# Autodesk Inventor assembly: 조립
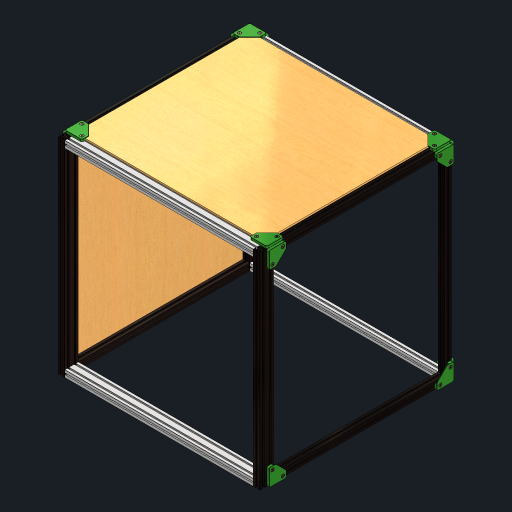
[picture p0: Inventor's stored thumbnail of the model, 512x512]
Saved by Autodesk Inventor 2024.1 (Build 281209000, 209)
## iProperties
Created: 2024-01-11
Part Number: 조립
Document SubType Name: Assembly
Designer: KBU
Author: KBU
## Documents named in this file (9)
- C:\Users\likek\Videos\Modeling\챔버\조립.iam
- C:\Users\likek\Videos\Modeling\챔버\600mm 20x20 Profile.ipt
- C:\Users\likek\Videos\Modeling\챔버\600mm 20x40 profile.ipt
- C:\Users\likek\Videos\Modeling\챔버\500mm 20x20 Profile.ipt
- C:\Users\likek\Videos\Modeling\챔버\모서리 결합 조립.iam
- C:\Users\likek\Videos\Modeling\챔버\510x570 패널.ipt
- C:\Users\likek\Videos\Modeling\챔버\550mm 20x40 profile.ipt
- C:\Users\likek\Videos\Modeling\챔버\550mm 20x20 Profile.ipt
- C:\Users\likek\Videos\Modeling\챔버\550x510 패널.ipt
## Components (31 placed, 8 different names)
1. 600mm 20x40 profile:1 — 플러쉬:12, 메이트:8, 플러쉬:13, 메이트:13, 플러쉬:23, 플러쉬:24, 메이트:46, 플러쉬:58, 플러쉬:59, 플러쉬:62, 플러쉬:63
2. 600mm 20x40 profile:2 — 플러쉬:6, 메이트:5, 플러쉬:7, 메이트:14, 메이트:18, 플러쉬:60, 플러쉬:61, 메이트:48
3. 500mm 20x20 Profile:1 — 플러쉬:6, 메이트:5, 플러쉬:7, 플러쉬:8, 플러쉬:9, 메이트:6, 플러쉬:31, 플러쉬:33, 플러쉬:34, 메이트:47, 메이트:50
4. 600mm 20x20 Profile:2 — 플러쉬:8, 플러쉬:9, 메이트:6, 메이트:11, 플러쉬:18, 플러쉬:19, 플러쉬:29, 메이트:16, 플러쉬:32, 메이트:17, 플러쉬:52, 메이트:42, 메이트:45, 플러쉬:57, 플러쉬:70
5. 500mm 20x20 Profile:2 — 플러쉬:12, 메이트:8, 플러쉬:13, 플러쉬:39, 메이트:25, 플러쉬:41, 플러쉬:42, 플러쉬:67
6. 600mm 20x20 Profile:3 — 플러쉬:35, 메이트:24, 플러쉬:40, 메이트:44, 플러쉬:55, 메이트:49, 플러쉬:65, 플러쉬:66, 메이트:52
7. 500mm 20x20 Profile:3 — 메이트:11, 플러쉬:18, 플러쉬:19, 플러쉬:25, 플러쉬:26, 플러쉬:30, 메이트:30, 플러쉬:45, 플러쉬:48, 메이트:35, 메이트:51
8. 500mm 20x20 Profile:4 — 메이트:13, 플러쉬:23, 플러쉬:24, 플러쉬:36, 메이트:22, 메이트:23, 플러쉬:37, 플러쉬:38, 메이트:29, 플러쉬:43, 플러쉬:50, 플러쉬:54, 플러쉬:64, 메이트:53
9. 모서리 결합 조립:1 [sub-assembly] — 플러쉬:25, 플러쉬:26, 메이트:14, 플러쉬:69
10. 모서리 결합 조립:2 [sub-assembly] — 플러쉬:29, 플러쉬:30, 메이트:16, 메이트:33, 메이트:34, 플러쉬:71
11. 모서리 결합 조립:3 [sub-assembly] — 플러쉬:31, 플러쉬:32, 메이트:17, 플러쉬:72
12. 모서리 결합 조립:4 [sub-assembly] — 플러쉬:33, 플러쉬:34, 메이트:18
13. 모서리 결합 조립:5 [sub-assembly] — 플러쉬:35, 플러쉬:36, 메이트:22, 메이트:36, 메이트:38, 플러쉬:74
14. 모서리 결합 조립:6 [sub-assembly] — 메이트:23, 플러쉬:37, 플러쉬:38, 플러쉬:68
15. 모서리 결합 조립:7 [sub-assembly] — 메이트:24, 플러쉬:39, 플러쉬:40, 메이트:37, 플러쉬:73
16. 모서리 결합 조립:8 [sub-assembly] — 메이트:25, 플러쉬:41, 플러쉬:42
17. 모서리 결합 조립:9 [sub-assembly] — 메이트:29, 플러쉬:43, 플러쉬:68, 메이트:56
18. 모서리 결합 조립:10 [sub-assembly] — 메이트:30, 플러쉬:45, 플러쉬:69
19. 모서리 결합 조립:11 [sub-assembly] — 플러쉬:48, 플러쉬:70, 메이트:51
20. 모서리 결합 조립:12 [sub-assembly] — 플러쉬:50, 플러쉬:75, 메이트:53, 메이트:54, 메이트:55
21. 510x570 패널:1 — 메이트:33, 메이트:34, 메이트:35
22. 510x570 패널:2 — 메이트:36, 메이트:37, 메이트:38
23. 모서리 결합 조립:13 [sub-assembly] — 플러쉬:52, 메이트:42, 플러쉬:71
24. 모서리 결합 조립:14 [sub-assembly] — 플러쉬:54, 플러쉬:74, 메이트:52
25. 모서리 결합 조립:15 [sub-assembly] — 메이트:44, 플러쉬:55, 플러쉬:73
26. 모서리 결합 조립:16 [sub-assembly] — 메이트:45, 플러쉬:57, 플러쉬:72
27. 550mm 20x40 profile:1 — 메이트:46, 플러쉬:58, 플러쉬:59, 플러쉬:60, 플러쉬:61, 메이트:47
28. 550mm 20x40 profile:2 — 플러쉬:62, 메이트:48, 플러쉬:63
29. 550mm 20x20 Profile:1 — 메이트:49, 플러쉬:64, 플러쉬:65, 플러쉬:75
30. 550mm 20x20 Profile:2 — 플러쉬:66, 플러쉬:67, 메이트:50
31. 550x510 패널:1 — 메이트:54, 메이트:55, 메이트:56
## Relationships (90: Flush 54, Mate 36)
- 플러쉬:6 [Flush]: 600mm 20x40 profile:2 ↔ 500mm 20x20 Profile:1
- 메이트:5 [Mate]: 600mm 20x40 profile:2 ↔ 500mm 20x20 Profile:1
- 플러쉬:7 [Flush]: 600mm 20x40 profile:2 ↔ 500mm 20x20 Profile:1
- 플러쉬:8 [Flush]: 500mm 20x20 Profile:1 ↔ 600mm 20x20 Profile:2
- 플러쉬:9 [Flush]: 500mm 20x20 Profile:1 ↔ 600mm 20x20 Profile:2
- 메이트:6 [Mate]: 500mm 20x20 Profile:1 ↔ 600mm 20x20 Profile:2
- [Flush]: 500mm 20x20 Profile:2 ↔ 600mm 20x20 Profile:3
- [Flush]: 500mm 20x20 Profile:2 ↔ 600mm 20x20 Profile:3
- [Mate]: 500mm 20x20 Profile:2 ↔ 600mm 20x20 Profile:3
- 플러쉬:12 [Flush]: 600mm 20x40 profile:1 ↔ 500mm 20x20 Profile:2
- 메이트:8 [Mate]: 600mm 20x40 profile:1 ↔ 500mm 20x20 Profile:2
- 플러쉬:13 [Flush]: 600mm 20x40 profile:1 ↔ 500mm 20x20 Profile:2
- 메이트:11 [Mate]: 600mm 20x20 Profile:2 ↔ 500mm 20x20 Profile:3
- 플러쉬:18 [Flush]: 600mm 20x20 Profile:2 ↔ 500mm 20x20 Profile:3
- 플러쉬:19 [Flush]: 600mm 20x20 Profile:2 ↔ 500mm 20x20 Profile:3
- 메이트:13 [Mate]: 600mm 20x40 profile:1 ↔ 500mm 20x20 Profile:4
- 플러쉬:23 [Flush]: 600mm 20x40 profile:1 ↔ 500mm 20x20 Profile:4
- 플러쉬:24 [Flush]: 600mm 20x40 profile:1 ↔ 500mm 20x20 Profile:4
- 플러쉬:25 [Flush]: 500mm 20x20 Profile:3 ↔ 모서리 결합 조립:1
- 플러쉬:26 [Flush] (-20 mm): 500mm 20x20 Profile:3 ↔ 모서리 결합 조립:1
- 메이트:14 [Mate]: 600mm 20x40 profile:2 ↔ 모서리 결합 조립:1
- 플러쉬:29 [Flush]: 600mm 20x20 Profile:2 ↔ 모서리 결합 조립:2
- 플러쉬:30 [Flush]: 500mm 20x20 Profile:3 ↔ 모서리 결합 조립:2
- 메이트:16 [Mate]: 600mm 20x20 Profile:2 ↔ 모서리 결합 조립:2
- 플러쉬:31 [Flush]: 500mm 20x20 Profile:1 ↔ 모서리 결합 조립:3
- 플러쉬:32 [Flush]: 600mm 20x20 Profile:2 ↔ 모서리 결합 조립:3
- 메이트:17 [Mate]: 600mm 20x20 Profile:2 ↔ 모서리 결합 조립:3
- 플러쉬:33 [Flush]: 500mm 20x20 Profile:1 ↔ 모서리 결합 조립:4
- 플러쉬:34 [Flush] (-20 mm): 500mm 20x20 Profile:1 ↔ 모서리 결합 조립:4
- 메이트:18 [Mate]: 600mm 20x40 profile:2 ↔ 모서리 결합 조립:4
- 플러쉬:35 [Flush]: 600mm 20x20 Profile:3 ↔ 모서리 결합 조립:5
- 플러쉬:36 [Flush]: 500mm 20x20 Profile:4 ↔ 모서리 결합 조립:5
- 메이트:22 [Mate]: 500mm 20x20 Profile:4 ↔ 모서리 결합 조립:5
- 메이트:23 [Mate]: 500mm 20x20 Profile:4 ↔ 모서리 결합 조립:6
- 플러쉬:37 [Flush]: 500mm 20x20 Profile:4 ↔ 모서리 결합 조립:6
- 플러쉬:38 [Flush] (-20 mm): 500mm 20x20 Profile:4 ↔ 모서리 결합 조립:6
- 메이트:24 [Mate]: 600mm 20x20 Profile:3 ↔ 모서리 결합 조립:7
- 플러쉬:39 [Flush]: 500mm 20x20 Profile:2 ↔ 모서리 결합 조립:7
- 플러쉬:40 [Flush]: 600mm 20x20 Profile:3 ↔ 모서리 결합 조립:7
- 메이트:25 [Mate]: 500mm 20x20 Profile:2 ↔ 모서리 결합 조립:8
- 플러쉬:41 [Flush]: 500mm 20x20 Profile:2 ↔ 모서리 결합 조립:8
- 플러쉬:42 [Flush] (-20 mm): 500mm 20x20 Profile:2 ↔ 모서리 결합 조립:8
- 메이트:29 [Mate]: 500mm 20x20 Profile:4 ↔ 모서리 결합 조립:9
- 플러쉬:43 [Flush]: 500mm 20x20 Profile:4 ↔ 모서리 결합 조립:9
- 메이트:30 [Mate]: 500mm 20x20 Profile:3 ↔ 모서리 결합 조립:10
- 플러쉬:45 [Flush]: 500mm 20x20 Profile:3 ↔ 모서리 결합 조립:10
- 플러쉬:48 [Flush]: 500mm 20x20 Profile:3 ↔ 모서리 결합 조립:11
- 플러쉬:50 [Flush]: 500mm 20x20 Profile:4 ↔ 모서리 결합 조립:12
- 메이트:33 [Mate] (1.5 mm): 모서리 결합 조립:2 ↔ 510x570 패널:1
- 메이트:34 [Mate] (1.5 mm): 모서리 결합 조립:2 ↔ 510x570 패널:1
- 메이트:35 [Mate] (0.15 mm): 500mm 20x20 Profile:3 ↔ 510x570 패널:1
- 메이트:36 [Mate] (1.5 mm): 모서리 결합 조립:5 ↔ 510x570 패널:2
- 메이트:37 [Mate] (1.5 mm): 모서리 결합 조립:7 ↔ 510x570 패널:2
- 메이트:38 [Mate] (0.15 mm): 모서리 결합 조립:5 ↔ 510x570 패널:2
- 플러쉬:52 [Flush]: 600mm 20x20 Profile:2 ↔ 모서리 결합 조립:13
- 메이트:42 [Mate]: 600mm 20x20 Profile:2 ↔ 모서리 결합 조립:13
- 플러쉬:54 [Flush]: 500mm 20x20 Profile:4 ↔ 모서리 결합 조립:14
- 메이트:44 [Mate]: 600mm 20x20 Profile:3 ↔ 모서리 결합 조립:15
- 플러쉬:55 [Flush]: 600mm 20x20 Profile:3 ↔ 모서리 결합 조립:15
- 메이트:45 [Mate]: 600mm 20x20 Profile:2 ↔ 모서리 결합 조립:16
- 플러쉬:57 [Flush]: 600mm 20x20 Profile:2 ↔ 모서리 결합 조립:16
- 메이트:46 [Mate]: 600mm 20x40 profile:1 ↔ 550mm 20x40 profile:1
- 플러쉬:58 [Flush]: 600mm 20x40 profile:1 ↔ 550mm 20x40 profile:1
- 플러쉬:59 [Flush]: 600mm 20x40 profile:1 ↔ 550mm 20x40 profile:1
- 플러쉬:60 [Flush]: 600mm 20x40 profile:2 ↔ 550mm 20x40 profile:1
- 플러쉬:61 [Flush]: 600mm 20x40 profile:2 ↔ 550mm 20x40 profile:1
- 메이트:47 [Mate]: 500mm 20x20 Profile:1 ↔ 550mm 20x40 profile:1
- 플러쉬:62 [Flush]: 600mm 20x40 profile:1 ↔ 550mm 20x40 profile:2
- 메이트:48 [Mate]: 600mm 20x40 profile:2 ↔ 550mm 20x40 profile:2
- 플러쉬:63 [Flush]: 600mm 20x40 profile:1 ↔ 550mm 20x40 profile:2
- 메이트:49 [Mate]: 600mm 20x20 Profile:3 ↔ 550mm 20x20 Profile:1
- 플러쉬:64 [Flush]: 500mm 20x20 Profile:4 ↔ 550mm 20x20 Profile:1
- 플러쉬:65 [Flush]: 600mm 20x20 Profile:3 ↔ 550mm 20x20 Profile:1
- 플러쉬:66 [Flush]: 600mm 20x20 Profile:3 ↔ 550mm 20x20 Profile:2
- 플러쉬:67 [Flush]: 500mm 20x20 Profile:2 ↔ 550mm 20x20 Profile:2
- 메이트:50 [Mate]: 500mm 20x20 Profile:1 ↔ 550mm 20x20 Profile:2
- 플러쉬:68 [Flush]: 모서리 결합 조립:6 ↔ 모서리 결합 조립:9
- 플러쉬:69 [Flush]: 모서리 결합 조립:1 ↔ 모서리 결합 조립:10
- 플러쉬:70 [Flush]: 600mm 20x20 Profile:2 ↔ 모서리 결합 조립:11
- 메이트:51 [Mate]: 500mm 20x20 Profile:3 ↔ 모서리 결합 조립:11
- 플러쉬:71 [Flush]: 모서리 결합 조립:2 ↔ 모서리 결합 조립:13
- 플러쉬:72 [Flush]: 모서리 결합 조립:3 ↔ 모서리 결합 조립:16
- 플러쉬:73 [Flush]: 모서리 결합 조립:7 ↔ 모서리 결합 조립:15
- 플러쉬:74 [Flush]: 모서리 결합 조립:5 ↔ 모서리 결합 조립:14
- 메이트:52 [Mate]: 600mm 20x20 Profile:3 ↔ 모서리 결합 조립:14
- 플러쉬:75 [Flush]: 모서리 결합 조립:12 ↔ 550mm 20x20 Profile:1
- 메이트:53 [Mate]: 500mm 20x20 Profile:4 ↔ 모서리 결합 조립:12
- 메이트:54 [Mate] (6 mm): 모서리 결합 조립:12 ↔ 550x510 패널:1
- 메이트:55 [Mate] (6 mm): 모서리 결합 조립:12 ↔ 550x510 패널:1
- 메이트:56 [Mate] (0.25 mm): 모서리 결합 조립:9 ↔ 550x510 패널:1
## Named parameters: d125_d122 = 0 mm, d126_d123 = 0 mm, d127_d124 = 0 mm
